# Autodesk Inventor assembly: Assembly1
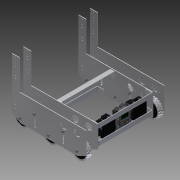
[picture p0: Inventor's stored thumbnail of the model, 180x180]
Saved by Autodesk Inventor 2014 (Build 180170000, 170)
## iProperties
Created: 2013-10-21
Part Number: Assembly1
Document SubType Name: Assembly
Designer: 14hensgenw
Author: 14hensgenw
## Documents named in this file (9)
- G:\!LANlords\V1\Assembly1.iam
- G:\!LANlords\V1\Side-Wall - 2014.ipt
- G:\!LANlords\V1\LANcrossmember.ipt
- G:\!LANlords\V1\tetrix_991445_2012.ipt
- G:\!LANlords\V1\nxt_brick_2012.iam
- G:\!LANlords\V1\tetrix_739102_2012.ipt
- G:\!LANlords\V1\1in standoff.ipt
- G:\FTC\4 in HiGrip Wheel.iam
- C:\Users\Wren\Documents\Inventor\Content Center Files\R2014\en-US\ANSI ASME B18.2.1(2)\ANSI_ASME B18.2.1 - 5_16-18 UNC - 3.25(2).ipt
## Components (34 placed, 8 different names)
1. Side-Wall - 2014:1 — Flush:2, Flush:4, Mate:2, Mate:36, Mate:37, Mate:38, Mate:39, Insert:1, Insert:2, Insert:3, Insert:4, Insert:6
2. Side-Wall - 2014:2 — Flush:2, Flush:3, Flush:4, Flush:5, Mate:2, Mate:3, Mate:5, Flush:10, Mate:9, Mate:15, Mate:17, Mate:40, Mate:41
3. Side-Wall - 2014:3 — Flush:1, Flush:3, Flush:5, Flush:6, Mate:1, Mate:4, Mate:7, Flush:8, Flush:9, Flush:11, Flush:12, Flush:13, Flush:14, Mate:10, Mate:16, Mate:31, Mate:33
4. Side-Wall - 2014:4 — Flush:1, Flush:6, Mate:1, Mate:30, Mate:32, Mate:34, Mate:35, Insert:8, Insert:9, Insert:11, Insert:13, Insert:14
5. LANcrossmember:1 — Mate:7, Flush:9
6. LANcrossmember:3 — Mate:5, Flush:13, Flush:14, Flush:15, Flush:16, Mate:11, Mate:12, Mate:13, Mate:14, Flush:18
7. LANcrossmember:4 — Mate:3, Mate:4, Flush:8, Flush:11
8. LANcrossmember:5 — Flush:10, Mate:9, Flush:12
9. LANcrossmember:6 — Mate:10, Flush:15, Flush:16
10. tetrix_991445_2012:1 — Mate:11, Mate:12, Flush:17, Mate:16, Mate:18, Mate:19, Flush:19, Mate:22, Mate:23
11. tetrix_991445_2012:4 — Flush:17, Mate:13, Mate:15, Mate:24, Flush:20, Flush:21, Mate:25, Mate:27
12. nxt_brick_2012:1 [sub-assembly] — Mate:14, Mate:17, Flush:18
13. tetrix_739102_2012:1 — Mate:18, Mate:19, Mate:20, Mate:21
14. tetrix_991445_2012:5 — Mate:20, Flush:19, Mate:21
15. tetrix_991445_2012:6 — Flush:20, Flush:21, Mate:26, Mate:28, Mate:29
16. 1in standoff:1 — Mate:27, Mate:28
17. 1in standoff:2 — Mate:22, Mate:23
18. 1in standoff:3 — Mate:24, Mate:25, Mate:26, Mate:29
19. 4 in HiGrip Wheel:1 [sub-assembly] — Mate:37, Mate:41
20. 4 in HiGrip Wheel:2 [sub-assembly] — Mate:30, Mate:31
21. 4 in HiGrip Wheel:3 [sub-assembly] — Mate:36, Mate:40
22. 4 in HiGrip Wheel:4 [sub-assembly] — Mate:32, Mate:33
23. 4 in HiGrip Wheel:5 [sub-assembly] — Mate:34, Mate:35
24. 4 in HiGrip Wheel:6 [sub-assembly] — Mate:38, Mate:39
25. Hex Bolt - Inch 5/16-18 UNC - 3.25:1 — Insert:1
26. Hex Bolt - Inch 5/16-18 UNC - 3.25:2 — Insert:2
27. Hex Bolt - Inch 5/16-18 UNC - 3.25:3 — Insert:3
28. Hex Bolt - Inch 5/16-18 UNC - 3.25:4 — Insert:4
29. Hex Bolt - Inch 5/16-18 UNC - 3.25:6 — Insert:6
30. Hex Bolt - Inch 5/16-18 UNC - 3.25:8 — Insert:8
31. Hex Bolt - Inch 5/16-18 UNC - 3.25:9 — Insert:9
32. Hex Bolt - Inch 5/16-18 UNC - 3.25:11 — Insert:11
33. Hex Bolt - Inch 5/16-18 UNC - 3.25:13 — Insert:13
34. Hex Bolt - Inch 5/16-18 UNC - 3.25:14 — Insert:14
## Relationships (69: Mate 39, Flush 20, Insert 10)
- Flush:1: Side-Wall - 2014:3 ↔ Side-Wall - 2014:4
- Flush:2: Side-Wall - 2014:1 ↔ Side-Wall - 2014:2
- Flush:3: Side-Wall - 2014:2 ↔ Side-Wall - 2014:3
- Flush:4: Side-Wall - 2014:1 ↔ Side-Wall - 2014:2
- Flush:5: Side-Wall - 2014:2 ↔ Side-Wall - 2014:3
- Flush:6: Side-Wall - 2014:3 ↔ Side-Wall - 2014:4
- Mate:1 (63.5 mm): Side-Wall - 2014:3 ↔ Side-Wall - 2014:4
- Mate:2 (63.5 mm): Side-Wall - 2014:1 ↔ Side-Wall - 2014:2
- Mate:3: Side-Wall - 2014:2 ↔ LANcrossmember:4
- Mate:4: Side-Wall - 2014:3 ↔ LANcrossmember:4
- Mate:5: Side-Wall - 2014:2 ↔ LANcrossmember:3
- Mate:7: Side-Wall - 2014:3 ↔ LANcrossmember:1
- Flush:8: Side-Wall - 2014:3 ↔ LANcrossmember:4
- Flush:9: Side-Wall - 2014:3 ↔ LANcrossmember:1
- Flush:10: Side-Wall - 2014:2 ↔ LANcrossmember:5
- Mate:9: Side-Wall - 2014:2 ↔ LANcrossmember:5
- Flush:11 (114.3 mm): Side-Wall - 2014:3 ↔ LANcrossmember:4
- Flush:12 (215.9 mm): Side-Wall - 2014:3 ↔ LANcrossmember:5
- Flush:13: Side-Wall - 2014:3 ↔ LANcrossmember:3
- Flush:14: Side-Wall - 2014:3 ↔ LANcrossmember:3
- Mate:10: Side-Wall - 2014:3 ↔ LANcrossmember:6
- Flush:15: LANcrossmember:3 ↔ LANcrossmember:6
- Flush:16 (88.9 mm): LANcrossmember:3 ↔ LANcrossmember:6
- Mate:11: LANcrossmember:3 ↔ tetrix_991445_2012:1
- Mate:12: LANcrossmember:3 ↔ tetrix_991445_2012:1
- Flush:17: tetrix_991445_2012:1 ↔ tetrix_991445_2012:4
- Mate:13: LANcrossmember:3 ↔ tetrix_991445_2012:4
- Mate:14: LANcrossmember:3 ↔ nxt_brick_2012:1
- Mate:15 (31.75 mm): Side-Wall - 2014:2 ↔ tetrix_991445_2012:4
- Mate:16 (31.75 mm): Side-Wall - 2014:3 ↔ tetrix_991445_2012:1
- Mate:17 (127 mm): Side-Wall - 2014:2 ↔ nxt_brick_2012:1
- Flush:18: LANcrossmember:3 ↔ nxt_brick_2012:1
- Mate:18: tetrix_991445_2012:1 ↔ tetrix_739102_2012:1
- Mate:19: tetrix_991445_2012:1 ↔ tetrix_739102_2012:1
- Mate:20: tetrix_739102_2012:1 ↔ tetrix_991445_2012:5
- Flush:19: tetrix_991445_2012:1 ↔ tetrix_991445_2012:5
- Mate:21: tetrix_739102_2012:1 ↔ tetrix_991445_2012:5
- Mate:22: tetrix_991445_2012:1 ↔ 1in standoff:2
- Mate:23: tetrix_991445_2012:1 ↔ 1in standoff:2
- Mate:24: tetrix_991445_2012:4 ↔ 1in standoff:3
- Flush:20: tetrix_991445_2012:4 ↔ tetrix_991445_2012:6
- Flush:21: tetrix_991445_2012:4 ↔ tetrix_991445_2012:6
- Mate:25: tetrix_991445_2012:4 ↔ 1in standoff:3
- Mate:26: tetrix_991445_2012:6 ↔ 1in standoff:3
- Mate:27: tetrix_991445_2012:4 ↔ 1in standoff:1
- Mate:28: tetrix_991445_2012:6 ↔ 1in standoff:1
- Mate:29: tetrix_991445_2012:6 ↔ 1in standoff:3
- Mate:30: Side-Wall - 2014:4 ↔ 4 in HiGrip Wheel:2
- Mate:31: Side-Wall - 2014:3 ↔ 4 in HiGrip Wheel:2
- Mate:32: Side-Wall - 2014:4 ↔ 4 in HiGrip Wheel:4
- Mate:33: Side-Wall - 2014:3 ↔ 4 in HiGrip Wheel:4
- Mate:34: Side-Wall - 2014:4 ↔ 4 in HiGrip Wheel:5
- Mate:35: Side-Wall - 2014:4 ↔ 4 in HiGrip Wheel:5
- Mate:36: Side-Wall - 2014:1 ↔ 4 in HiGrip Wheel:3
- Mate:37: Side-Wall - 2014:1 ↔ 4 in HiGrip Wheel:1
- Mate:38: Side-Wall - 2014:1 ↔ 4 in HiGrip Wheel:6
- Mate:39: Side-Wall - 2014:1 ↔ 4 in HiGrip Wheel:6
- Mate:40: Side-Wall - 2014:2 ↔ 4 in HiGrip Wheel:3
- Mate:41: Side-Wall - 2014:2 ↔ 4 in HiGrip Wheel:1
- Insert:1 (-81.7104 mm): Side-Wall - 2014:1 ↔ Hex Bolt - Inch 5/16-18 UNC - 3.25:1
- Insert:2 (-81.7104 mm): Side-Wall - 2014:1 ↔ Hex Bolt - Inch 5/16-18 UNC - 3.25:2
- Insert:3 (-81.7104 mm): Side-Wall - 2014:1 ↔ Hex Bolt - Inch 5/16-18 UNC - 3.25:3
- Insert:4 (-81.7104 mm): Side-Wall - 2014:1 ↔ Hex Bolt - Inch 5/16-18 UNC - 3.25:4
- Insert:6 (-81.7104 mm): Side-Wall - 2014:1 ↔ Hex Bolt - Inch 5/16-18 UNC - 3.25:6
- Insert:8 (-81.7104 mm): Side-Wall - 2014:4 ↔ Hex Bolt - Inch 5/16-18 UNC - 3.25:8
- Insert:9 (-81.7104 mm): Side-Wall - 2014:4 ↔ Hex Bolt - Inch 5/16-18 UNC - 3.25:9
- Insert:11 (-81.7104 mm): Side-Wall - 2014:4 ↔ Hex Bolt - Inch 5/16-18 UNC - 3.25:11
- Insert:13 (-81.7104 mm): Side-Wall - 2014:4 ↔ Hex Bolt - Inch 5/16-18 UNC - 3.25:13
- Insert:14 (-81.7104 mm): Side-Wall - 2014:4 ↔ Hex Bolt - Inch 5/16-18 UNC - 3.25:14
